# Autodesk Inventor assembly: Gear chain
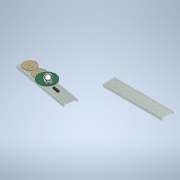
[picture p0: Inventor's stored thumbnail of the model, 180x180]
Saved by Autodesk Inventor 2021 (Build 250183000, 183)
## iProperties
Created: 2021-02-10
Part Number: Gear chain
Document SubType Name: Assembly
Designer: david
Author: david
## Documents named in this file (7)
- C:\Users\david\OneDrive\Documents\Inventor\Gear chain.iam
- C:\Users\david\OneDrive\Documents\Inventor\Inventor_2013_VEX_KOP_-_Imperial\Imperial\Motion\60 Tooth Gear.ipt
- C:\Users\david\OneDrive\Documents\Inventor\Inventor_2013_VEX_KOP_-_Imperial\Imperial\Motion\36 Tooth Gear.ipt
- C:\Users\david\OneDrive\Documents\Inventor\Inventor_2013_VEX_KOP_-_Imperial\Imperial\Motion\Shaft 2 inch.ipt
- C:\Users\david\OneDrive\Documents\Inventor\Inventor_2013_VEX_KOP_-_Imperial\Imperial\Motion\Bearing Flat.ipt
- C:\Users\david\OneDrive\Documents\Inventor\Inventor_2013_VEX_KOP_-_Imperial\Imperial\Structure\C-Channel 1x5x1x25 Hole.ipt
- C:\Users\david\OneDrive\Documents\Inventor\Inventor_2013_VEX_KOP_-_Imperial\Imperial\Motion\84 Tooth Gear.ipt
## Components (14 placed, 6 different names)
1. 60 Tooth Gear:1 — Insert:3, Insert:4
2. 60 Tooth Gear:2 — Insert:1, Insert:2
3. 36 Tooth Gear:1 — Insert:6, Insert:7
4. Shaft 2 inch:1 — Insert:1, Mate:9
5. Bearing Flat:1 — Insert:2, Mate:1, Mate:2
6. C-Channel 1x5x1x25 Hole:1 — Mate:1, Mate:2, Mate:3, Mate:4, Mate:5, Mate:6, Mate:7, Mate:8, Mate:9, Mate:10, Mate:11
7. C-Channel 1x5x1x25 Hole:2
8. Bearing Flat:2 — Insert:4, Mate:3, Mate:4
9. Bearing Flat:3 — Insert:6, Mate:5, Mate:6
10. Bearing Flat:4 — Mate:10, Mate:11
11. Shaft 2 inch:2
12. Shaft 2 inch:3 — Insert:3, Mate:8
13. Shaft 2 inch:4 — Mate:7
14. 84 Tooth Gear:1 — Insert:7
## Relationships (17: Mate 11, Insert 6)
- Insert:1: 60 Tooth Gear:2 ↔ Shaft 2 inch:1
- Insert:2: 60 Tooth Gear:2 ↔ Bearing Flat:1
- Mate:1: Bearing Flat:1 ↔ C-Channel 1x5x1x25 Hole:1
- Mate:2: Bearing Flat:1 ↔ C-Channel 1x5x1x25 Hole:1
- Insert:3: 60 Tooth Gear:1 ↔ Shaft 2 inch:3
- Insert:4: 60 Tooth Gear:1 ↔ Bearing Flat:2
- Mate:3: C-Channel 1x5x1x25 Hole:1 ↔ Bearing Flat:2
- Mate:4: C-Channel 1x5x1x25 Hole:1 ↔ Bearing Flat:2
- Insert:6: 36 Tooth Gear:1 ↔ Bearing Flat:3
- Mate:5: C-Channel 1x5x1x25 Hole:1 ↔ Bearing Flat:3
- Mate:6: C-Channel 1x5x1x25 Hole:1 ↔ Bearing Flat:3
- Mate:7: C-Channel 1x5x1x25 Hole:1 ↔ Shaft 2 inch:4
- Mate:8: C-Channel 1x5x1x25 Hole:1 ↔ Shaft 2 inch:3
- Mate:9: Shaft 2 inch:1 ↔ C-Channel 1x5x1x25 Hole:1
- Mate:10: C-Channel 1x5x1x25 Hole:1 ↔ Bearing Flat:4
- Mate:11: C-Channel 1x5x1x25 Hole:1 ↔ Bearing Flat:4
- Insert:7: 36 Tooth Gear:1 ↔ 84 Tooth Gear:1
